# Autodesk Inventor assembly: snap_mount
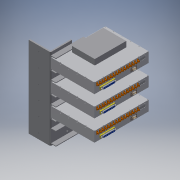
[picture p0: Inventor's stored thumbnail of the model, 180x180]
Saved by Autodesk Inventor 2017 (Build 210142000, 142)
## iProperties
Created: 2018-03-08
Part Number: snap_mount
Document SubType Name: Assembly
Designer: Zara
Author: Zara
## Documents named in this file (5)
- C:\Users\Zara\Documents\hera-cad\Node\SNAP_mount\snap_mount.iam
- C:\Users\Zara\Documents\hera-cad\Node\SNAP_mount\ubracket.ipt
- C:\Users\Zara\Documents\hera-cad\Node\SNAP_mount\uchannel.ipt
- C:\Users\Zara\Documents\hera-cad\Node\SNAP_V2\Workspaces\Workspace\SNAP 8x10x1.75 Ver1.A.iam
- C:\Users\Zara\Documents\hera-cad\Node\SNAP_mount\outer_heatsink.ipt
## Components (13 placed, 4 different names)
1. ubracket:1 — Mate:3, Flush:3, Mate:6, Mate:7, Mate:8, Mate:9, Mate:10, Mate:11, Mate:12, Mate:13
2. uchannel:1 — Mate:1, Flush:1, Mate:2, Mate:3, Mate:5, Mate:6, Mate:7
3. SNAP 8x10x1.75 Ver1.A:1 [sub-assembly] — Mate:1, Flush:1, Mate:2, Mate:4, Flush:2, Flush:3
4. outer_heatsink:1 — Mate:4, Flush:2, Mate:5
5. uchannel:2 — Mate:8, Mate:9
6. SNAP 8x10x1.75 Ver1.A:2 [sub-assembly]
7. outer_heatsink:2
8. uchannel:3 — Mate:10, Mate:11
9. SNAP 8x10x1.75 Ver1.A:3 [sub-assembly]
10. outer_heatsink:3
11. uchannel:4 — Mate:12, Mate:13
12. SNAP 8x10x1.75 Ver1.A:4 [sub-assembly]
13. outer_heatsink:4
## Component patterns: (4 elements, first: uchannel:1 + SNAP 8x10x1.75 Ver1.A:1 + outer_heatsink:1)
## Relationships (16: Mate 13, Flush 3)
- Mate:1: uchannel:1 ↔ SNAP 8x10x1.75 Ver1.A:1
- Flush:1: uchannel:1 ↔ SNAP 8x10x1.75 Ver1.A:1
- Mate:2 (4.7244 mm): uchannel:1 ↔ SNAP 8x10x1.75 Ver1.A:1
- Mate:3: ubracket:1 ↔ uchannel:1
- Mate:4: SNAP 8x10x1.75 Ver1.A:1 ↔ outer_heatsink:1
- Flush:2 (69.85 mm): SNAP 8x10x1.75 Ver1.A:1 ↔ outer_heatsink:1
- Mate:5 (5.08 mm): uchannel:1 ↔ outer_heatsink:1
- Flush:3: ubracket:1 ↔ SNAP 8x10x1.75 Ver1.A:1
- Mate:6: ubracket:1 ↔ uchannel:1
- Mate:7: ubracket:1 ↔ uchannel:1
- Mate:8: ubracket:1 ↔ uchannel:2
- Mate:9: ubracket:1 ↔ uchannel:2
- Mate:10: ubracket:1 ↔ uchannel:3
- Mate:11: ubracket:1 ↔ uchannel:3
- Mate:12: ubracket:1 ↔ uchannel:4
- Mate:13: ubracket:1 ↔ uchannel:4
